# Autodesk Inventor assembly: 20170529_chassis_assembly
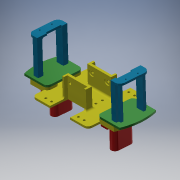
[picture p0: Inventor's stored thumbnail of the model, 180x180]
Saved by Autodesk Inventor 2017 SP1 (Build 210196100, 196)
## iProperties
Part Number: 20170529_chassis_assembly
Material: Générique
Document SubType Name: Assembly
Designer: tmonglon
Author: tmonglon
## Documents named in this file (5)
- D:\Inventor\Ahmet\design-20170821\design-20170821\design\chassis_assembly.iam
- D:\Inventor\Ahmet\design-20170821\design-20170821\design\red_part.ipt
- D:\Inventor\Ahmet\design-20170821\design-20170821\design\yellow_part.ipt
- D:\Inventor\Ahmet\design-20170821\design-20170821\design\green_part.ipt
- D:\Inventor\Ahmet\design-20170821\design-20170821\design\blue_part.ipt
## Components (6 placed, 4 different names)
1. red_part:1 — Logement:1, Placage:1
2. yellow_part:1 — Logement:1, Placage:1, Logement:2, Logement:3, Logement:4, Logement:5, Logement:6, Logement:8, Logement:9
3. green_part:1 — Logement:2, Logement:5, Logement:7
4. green_part:2 — Logement:3, Logement:4
5. blue_part:1 — Logement:6, Logement:7
6. blue_part:2 — Logement:8, Logement:9
## Relationships (10: Insert 9, Mate 1)
- Logement:1 [Insert]: red_part:1 ↔ yellow_part:1
- Placage:1 [Mate]: red_part:1 ↔ yellow_part:1
- Logement:2 [Insert]: yellow_part:1 ↔ green_part:1
- Logement:3 [Insert]: yellow_part:1 ↔ green_part:2
- Logement:4 [Insert]: yellow_part:1 ↔ green_part:2
- Logement:5 [Insert]: yellow_part:1 ↔ green_part:1
- Logement:6 [Insert]: yellow_part:1 ↔ blue_part:1
- Logement:7 [Insert]: green_part:1 ↔ blue_part:1
- Logement:8 [Insert]: yellow_part:1 ↔ blue_part:2
- Logement:9 [Insert]: yellow_part:1 ↔ blue_part:2
